# Autodesk Inventor assembly: Gantry Assembly R2
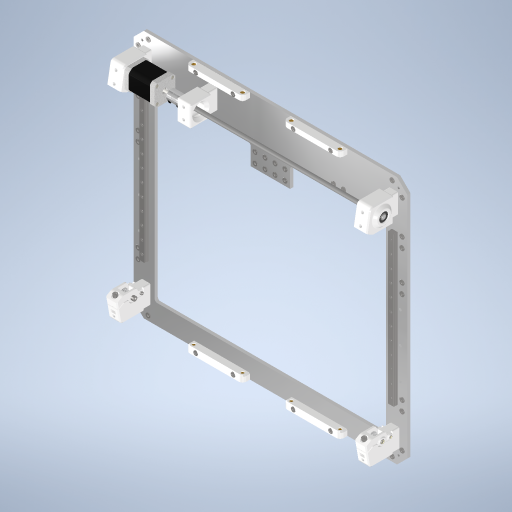
[picture p0: Inventor's stored thumbnail of the model, 512x512]
Saved by Autodesk Inventor 2024 (Build 280153000, 153)
## iProperties
Created: 2024-11-09
Part Number: Gantry Assembly R2
Document SubType Name: Assembly
Designer: Ishaan
Author: Ishaan
## Documents named in this file (24)
- E:\Projects\Axiom--IDEX-3D-Printer\CAD\04 - Gantry and Y-axis\Gantry Assembly R2.iam
- E:\Projects\Axiom--IDEX-3D-Printer\CAD\04 - Gantry and Y-axis\Printer Gantry Plate RevII.ipt
- E:\Projects\Axiom--IDEX-3D-Printer\CAD\00 - COTS Components\MGNR12 300mm Rail\MGNR12R100HM\MGNR12R100HM.ipt
- E:\Projects\Axiom--IDEX-3D-Printer\CAD\00 - COTS Components\Hardware\SHCSM3x8.ipt
- E:\Projects\Axiom--IDEX-3D-Printer\CAD\04 - Gantry and Y-axis\Y-axis Motor Block.ipt
- E:\Projects\Axiom--IDEX-3D-Printer\CAD\04 - Gantry and Y-axis\Y-axis Shaft Support.ipt
- E:\Projects\Axiom--IDEX-3D-Printer\CAD\04 - Gantry and Y-axis\Y-axis Bearing Pulley Block.ipt
- E:\Projects\Axiom--IDEX-3D-Printer\CAD\04 - Gantry and Y-axis\R2 Idler Block Left.ipt
- E:\Projects\Axiom--IDEX-3D-Printer\CAD\04 - Gantry and Y-axis\R2 Idler Block Right.ipt
- E:\Projects\Axiom--IDEX-3D-Printer\CAD\00 - COTS Components\NEMA 17 - Y-Axis\NEMA 17 Y-axis.ipt
- E:\Projects\Axiom--IDEX-3D-Printer\CAD\00 - COTS Components\9mm 20T GT2 Timing Pulley 5mm Bore\9mm 20T GT2 Timing Pulley 5mm Bore.ipt
- E:\Projects\Axiom--IDEX-3D-Printer\CAD\00 - COTS Components\9mm 20T GT2 Idler Pulley 5mm Bore\9mm 20T GT2 Idler Pulley 5mm Bore.ipt
- E:\Projects\Axiom--IDEX-3D-Printer\CAD\00 - COTS Components\608-2RS\608-2RS Bearing.ipt
- E:\Projects\Axiom--IDEX-3D-Printer\CAD\00 - COTS Components\9mm 20T GT2 Timing Pulley 8mm Bore\9mm 20T GT2 Timing Pulley 8mm Bore.ipt
- E:\Projects\Axiom--IDEX-3D-Printer\CAD\00 - COTS Components\5x8 Shaft Coupler\Flexible Coupling 5mm x 8mm.ipt
- E:\Projects\Axiom--IDEX-3D-Printer\CAD\00 - COTS Components\Hardware\SHCSM3x25.ipt
- E:\Projects\Axiom--IDEX-3D-Printer\CAD\00 - COTS Components\Hardware\SHCSM5x16.ipt
- E:\Projects\Axiom--IDEX-3D-Printer\CAD\00 - COTS Components\Hardware\Low Profile M5x12.ipt
- E:\Projects\Axiom--IDEX-3D-Printer\CAD\00 - COTS Components\Hardware\SHCSM5x25.ipt
- E:\Projects\Axiom--IDEX-3D-Printer\CAD\00 - COTS Components\Hardware\M5 LOCKNUT.ipt
- E:\Projects\Axiom--IDEX-3D-Printer\CAD\00 - COTS Components\Hardware\M3 LOCKNUT.ipt
- E:\Projects\Axiom--IDEX-3D-Printer\CAD\04 - Gantry and Y-axis\Y-axis Power Transfer Shaft 415mm.ipt
- E:\Projects\Axiom--IDEX-3D-Printer\CAD\04 - Gantry and Y-axis\Front Panel Mount.ipt
- E:\Projects\Axiom--IDEX-3D-Printer\CAD\00 - COTS Components\Hardware\M5 Heat Set Insert.ipt
## Components (118 placed, 23 different names)
1. Printer Gantry Plate RevII:1 — Insert:1, Insert:2, Insert:3, Insert:4, Insert:6, Insert:7, Insert:8, Insert:9, Insert:10, Insert:11, Insert:12, Insert:13, Insert:14, Insert:15, Insert:36, Insert:37, Insert:38, Insert:39, Insert:40, Insert:41, Insert:42, Insert:43, Insert:44, Insert:45, Insert:46, Insert:47, Insert:48, Insert:49, Insert:50, Insert:51, Insert:52, Insert:53, Insert:54, Insert:55, Insert:56, Insert:57, Insert:58, Insert:59, Insert:60, Insert:61, Insert:62, Insert:63, Insert:64, Insert:65, Insert:66, Insert:67, Insert:77, Insert:78, Insert:79, Insert:80, Insert:81, Insert:82, Insert:83, Insert:84
2. MGNR12R100HM:1 — Insert:3, Insert:4, Insert:5, Flush:3, Mate:4
3. MGNR12R100HM:2 — Insert:1, Insert:2, Flush:1, Flush:2, Insert:76
4. Y-axis Motor Block:1 — Insert:6, Insert:7, Insert:16, Insert:17, Insert:22, Insert:23, Insert:24, Insert:25, Insert:30, Insert:31
5. Y-axis Shaft Support:1 — Insert:8, Insert:9, Insert:18, Insert:32, Insert:33
6. Y-axis Bearing Pulley Block:1 — Insert:10, Insert:11, Insert:19, Insert:20, Insert:34, Insert:35
7. R2 Idler Block Left:1 — Insert:12, Insert:13, Mate:3, Insert:26, Insert:27, Insert:68, Mate:11, Mate:12, Insert:71, Insert:73, Angle:1, Insert:75, Angle:4
8. R2 Idler Block Right:1 — Insert:14, Insert:15, Mate:2, Insert:28, Insert:29, Insert:69, Mate:9, Mate:10, Insert:70, Insert:72, Angle:2, Insert:74, Angle:3
9. NEMA 17 Y-axis:1 — Insert:16, Insert:17, Mate:1, Insert:21
10. 9mm 20T GT2 Timing Pulley 5mm Bore:1 — Mate:1, Flush:1
11. 9mm 20T GT2 Idler Pulley 5mm Bore:1 — Mate:2, Flush:2
12. 9mm 20T GT2 Idler Pulley 5mm Bore:2 — Mate:3, Flush:3
13. 608-2RS Bearing:1 — Insert:18
14. 608-2RS Bearing:2 — Insert:20
15. 608-2RS Bearing:3 — Insert:19, Mate:5
16. 9mm 20T GT2 Timing Pulley 8mm Bore:1 — Mate:4, Mate:5
17. Y-axis Power Transfer Shaft 415mm:1
18. Flexible Coupling 5mm x 8mm:1 — Insert:21
19. Front Panel Mount:1 — Insert:77, Insert:79, Insert:85, Insert:86, Insert:94
20. Front Panel Mount:2 — Insert:78, Insert:80, Insert:87, Insert:88
21. Front Panel Mount:3 — Insert:81, Insert:82, Insert:91, Insert:92
22. Front Panel Mount:4 — Insert:83, Insert:84, Insert:89, Insert:90, Insert:93
23. SHCSM5x16:11 — Insert:85
24. SHCSM5x16:12 — Insert:86
25. SHCSM5x16:13 — Insert:87
26. SHCSM5x16:14 — Insert:88
27. SHCSM5x16:15 — Insert:89
28. SHCSM5x16:16 — Insert:90
29. SHCSM5x16:17 — Insert:91
30. SHCSM5x16:18 — Insert:92
31. SHCSM5x25:1 — Insert:68
32. SHCSM5x25:2 — Insert:69
33. SHCSM5x25:3 — Mate:9, Mate:10
34. SHCSM5x25:4 — Mate:11, Mate:12
35. SHCSM3x25:5 — Insert:70
36. SHCSM3x25:6 — Insert:71
37. M5 LOCKNUT:1 — Insert:72, Angle:2
38. M5 LOCKNUT:2 — Insert:73, Angle:1
39. M3 LOCKNUT:1 — Insert:74, Angle:3
40. M3 LOCKNUT:2 — Insert:75, Angle:4
41. Low Profile M5x12:1 — Insert:36
42. Low Profile M5x12:2 — Insert:37
43. Low Profile M5x12:3 — Insert:38
44. Low Profile M5x12:4 — Insert:39
45. Low Profile M5x12:5 — Insert:40
46. Low Profile M5x12:6 — Insert:41
47. Low Profile M5x12:7 — Insert:42
48. Low Profile M5x12:8 — Insert:43
49. Low Profile M5x12:9 — Insert:45
50. Low Profile M5x12:10 — Insert:46
51. Low Profile M5x12:11 — Insert:49
52. Low Profile M5x12:12 — Insert:50
53. Low Profile M5x12:13 — Insert:44
54. Low Profile M5x12:14 — Insert:47
55. Low Profile M5x12:15 — Insert:48
56. Low Profile M5x12:16 — Insert:51
57. Low Profile M5x12:17 — Insert:52
58. Low Profile M5x12:18 — Insert:53
59. Low Profile M5x12:19 — Insert:54
60. Low Profile M5x12:20 — Insert:55
61. Low Profile M5x12:21 — Insert:56
62. Low Profile M5x12:22 — Insert:57
63. Low Profile M5x12:23 — Insert:58
64. Low Profile M5x12:24 — Insert:59
65. Low Profile M5x12:25 — Insert:60
66. Low Profile M5x12:26 — Insert:61
67. Low Profile M5x12:27 — Insert:62
68. Low Profile M5x12:28 — Insert:63
69. Low Profile M5x12:29 — Insert:64
70. Low Profile M5x12:30 — Insert:65
71. Low Profile M5x12:31 — Insert:66
72. Low Profile M5x12:32 — Insert:67
73. SHCSM3x25:1 — Insert:22
74. SHCSM3x25:2 — Insert:23
75. SHCSM3x25:3 — Insert:24
76. SHCSM3x25:4 — Insert:25
77. SHCSM5x16:1 — Insert:26
78. SHCSM5x16:2 — Insert:27
79. SHCSM5x16:3 — Insert:28
80. SHCSM5x16:4 — Insert:29
81. SHCSM5x16:5 — Insert:30
82. SHCSM5x16:6 — Insert:31
83. SHCSM5x16:7 — Insert:32
84. SHCSM5x16:8 — Insert:33
85. SHCSM5x16:9 — Insert:34
86. SHCSM5x16:10 — Insert:35
87. M5 Heat Set Insert:2 — Insert:93
88. M5 Heat Set Insert:3
89. M5 Heat Set Insert:4
90. M5 Heat Set Insert:5
91. M5 Heat Set Insert:1 — Insert:94
92. M5 Heat Set Insert:6
93. M5 Heat Set Insert:7
94. M5 Heat Set Insert:8
95. SHCSM3x8:1 — Insert:76
96. SHCSM3x8:2
97. SHCSM3x8:3
98. SHCSM3x8:4
99. SHCSM3x8:5
100. SHCSM3x8:6
101. SHCSM3x8:7
102. SHCSM3x8:8
103. SHCSM3x8:9
104. SHCSM3x8:10
105. SHCSM3x8:11
106. SHCSM3x8:12
107. SHCSM3x8:13 — Insert:5
108. SHCSM3x8:14
109. SHCSM3x8:15
110. SHCSM3x8:16
111. SHCSM3x8:17
112. SHCSM3x8:18
113. SHCSM3x8:19
114. SHCSM3x8:20
115. SHCSM3x8:21
116. SHCSM3x8:22
117. SHCSM3x8:23
118. SHCSM3x8:24
## Component patterns: (4 elements, first: M5 Heat Set Insert:2), (4 elements, first: M5 Heat Set Insert:1), (12 elements, first: SHCSM3x8:1), (12 elements, first: SHCSM3x8:13)
## Relationships (113: Insert 94, Mate 12, Angle 4, Flush 3)
- Insert:1: Printer Gantry Plate RevII:1 ↔ MGNR12R100HM:2
- Insert:2: Printer Gantry Plate RevII:1 ↔ MGNR12R100HM:2
- Insert:3: Printer Gantry Plate RevII:1 ↔ MGNR12R100HM:1
- Insert:4: Printer Gantry Plate RevII:1 ↔ MGNR12R100HM:1
- Insert:5: MGNR12R100HM:1 ↔ SHCSM3x8:13
- Insert:6: Printer Gantry Plate RevII:1 ↔ Y-axis Motor Block:1
- Insert:7: Printer Gantry Plate RevII:1 ↔ Y-axis Motor Block:1
- Insert:8: Printer Gantry Plate RevII:1 ↔ Y-axis Shaft Support:1
- Insert:9: Printer Gantry Plate RevII:1 ↔ Y-axis Shaft Support:1
- Insert:10: Printer Gantry Plate RevII:1 ↔ Y-axis Bearing Pulley Block:1
- Insert:11: Printer Gantry Plate RevII:1 ↔ Y-axis Bearing Pulley Block:1
- Insert:12: Printer Gantry Plate RevII:1 ↔ R2 Idler Block Left:1
- Insert:13: Printer Gantry Plate RevII:1 ↔ R2 Idler Block Left:1
- Insert:14: Printer Gantry Plate RevII:1 ↔ R2 Idler Block Right:1
- Insert:15: Printer Gantry Plate RevII:1 ↔ R2 Idler Block Right:1
- Insert:16: Y-axis Motor Block:1 ↔ NEMA 17 Y-axis:1
- Insert:17: Y-axis Motor Block:1 ↔ NEMA 17 Y-axis:1
- Mate:1: NEMA 17 Y-axis:1 ↔ 9mm 20T GT2 Timing Pulley 5mm Bore:1
- Flush:1: MGNR12R100HM:2 ↔ 9mm 20T GT2 Timing Pulley 5mm Bore:1
- Mate:2: R2 Idler Block Right:1 ↔ 9mm 20T GT2 Idler Pulley 5mm Bore:1
- Mate:3: R2 Idler Block Left:1 ↔ 9mm 20T GT2 Idler Pulley 5mm Bore:2
- Flush:2: MGNR12R100HM:2 ↔ 9mm 20T GT2 Idler Pulley 5mm Bore:1
- Flush:3: MGNR12R100HM:1 ↔ 9mm 20T GT2 Idler Pulley 5mm Bore:2
- Insert:18: Y-axis Shaft Support:1 ↔ 608-2RS Bearing:1
- Insert:19: Y-axis Bearing Pulley Block:1 ↔ 608-2RS Bearing:3
- Insert:20: Y-axis Bearing Pulley Block:1 ↔ 608-2RS Bearing:2
- Mate:4: MGNR12R100HM:1 ↔ 9mm 20T GT2 Timing Pulley 8mm Bore:1
- Mate:5: 608-2RS Bearing:3 ↔ 9mm 20T GT2 Timing Pulley 8mm Bore:1
- [Mate]: 608-2RS Bearing:3 ↔ Y-axis Power Transfer Shaft 415mm:1
- [Mate]: 608-2RS Bearing:1 ↔ Y-axis Power Transfer Shaft 415mm:1
- [Mate] (1 mm): NEMA 17 Y-axis:1 ↔ Y-axis Power Transfer Shaft 415mm:1
- Insert:21 (-0.5 mm): NEMA 17 Y-axis:1 ↔ Flexible Coupling 5mm x 8mm:1
- Insert:22: Y-axis Motor Block:1 ↔ SHCSM3x25:1
- Insert:23: Y-axis Motor Block:1 ↔ SHCSM3x25:2
- Insert:24: Y-axis Motor Block:1 ↔ SHCSM3x25:3
- Insert:25: Y-axis Motor Block:1 ↔ SHCSM3x25:4
- Insert:26: R2 Idler Block Left:1 ↔ SHCSM5x16:1
- Insert:27: R2 Idler Block Left:1 ↔ SHCSM5x16:2
- Insert:28: R2 Idler Block Right:1 ↔ SHCSM5x16:3
- Insert:29: R2 Idler Block Right:1 ↔ SHCSM5x16:4
- Insert:30: Y-axis Motor Block:1 ↔ SHCSM5x16:5
- Insert:31: Y-axis Motor Block:1 ↔ SHCSM5x16:6
- Insert:32: Y-axis Shaft Support:1 ↔ SHCSM5x16:7
- Insert:33: Y-axis Shaft Support:1 ↔ SHCSM5x16:8
- Insert:34: Y-axis Bearing Pulley Block:1 ↔ SHCSM5x16:9
- Insert:35: Y-axis Bearing Pulley Block:1 ↔ SHCSM5x16:10
- Insert:36: Printer Gantry Plate RevII:1 ↔ Low Profile M5x12:1
- Insert:37: Printer Gantry Plate RevII:1 ↔ Low Profile M5x12:2
- Insert:38: Printer Gantry Plate RevII:1 ↔ Low Profile M5x12:3
- Insert:39: Printer Gantry Plate RevII:1 ↔ Low Profile M5x12:4
- Insert:40: Printer Gantry Plate RevII:1 ↔ Low Profile M5x12:5
- Insert:41: Printer Gantry Plate RevII:1 ↔ Low Profile M5x12:6
- Insert:42: Printer Gantry Plate RevII:1 ↔ Low Profile M5x12:7
- Insert:43: Printer Gantry Plate RevII:1 ↔ Low Profile M5x12:8
- Insert:44: Printer Gantry Plate RevII:1 ↔ Low Profile M5x12:13
- Insert:45: Printer Gantry Plate RevII:1 ↔ Low Profile M5x12:9
- Insert:46: Printer Gantry Plate RevII:1 ↔ Low Profile M5x12:10
- Insert:47: Printer Gantry Plate RevII:1 ↔ Low Profile M5x12:14
- Insert:48: Printer Gantry Plate RevII:1 ↔ Low Profile M5x12:15
- Insert:49: Printer Gantry Plate RevII:1 ↔ Low Profile M5x12:11
- Insert:50: Printer Gantry Plate RevII:1 ↔ Low Profile M5x12:12
- Insert:51: Printer Gantry Plate RevII:1 ↔ Low Profile M5x12:16
- Insert:52: Printer Gantry Plate RevII:1 ↔ Low Profile M5x12:17
- Insert:53: Printer Gantry Plate RevII:1 ↔ Low Profile M5x12:18
- Insert:54: Printer Gantry Plate RevII:1 ↔ Low Profile M5x12:19
- Insert:55: Printer Gantry Plate RevII:1 ↔ Low Profile M5x12:20
- Insert:56: Printer Gantry Plate RevII:1 ↔ Low Profile M5x12:21
- Insert:57: Printer Gantry Plate RevII:1 ↔ Low Profile M5x12:22
- Insert:58: Printer Gantry Plate RevII:1 ↔ Low Profile M5x12:23
- Insert:59: Printer Gantry Plate RevII:1 ↔ Low Profile M5x12:24
- Insert:60: Printer Gantry Plate RevII:1 ↔ Low Profile M5x12:25
- Insert:61: Printer Gantry Plate RevII:1 ↔ Low Profile M5x12:26
- Insert:62: Printer Gantry Plate RevII:1 ↔ Low Profile M5x12:27
- Insert:63: Printer Gantry Plate RevII:1 ↔ Low Profile M5x12:28
- Insert:64: Printer Gantry Plate RevII:1 ↔ Low Profile M5x12:29
- Insert:65: Printer Gantry Plate RevII:1 ↔ Low Profile M5x12:30
- Insert:66: Printer Gantry Plate RevII:1 ↔ Low Profile M5x12:31
- Insert:67: Printer Gantry Plate RevII:1 ↔ Low Profile M5x12:32
- Insert:68: R2 Idler Block Left:1 ↔ SHCSM5x25:1
- Insert:69: R2 Idler Block Right:1 ↔ SHCSM5x25:2
- Mate:9: R2 Idler Block Right:1 ↔ SHCSM5x25:3
- Mate:10: R2 Idler Block Right:1 ↔ SHCSM5x25:3
- Mate:11: R2 Idler Block Left:1 ↔ SHCSM5x25:4
- Mate:12: R2 Idler Block Left:1 ↔ SHCSM5x25:4
- Insert:70: R2 Idler Block Right:1 ↔ SHCSM3x25:5
- Insert:71: R2 Idler Block Left:1 ↔ SHCSM3x25:6
- Insert:72: R2 Idler Block Right:1 ↔ M5 LOCKNUT:1
- Insert:73: R2 Idler Block Left:1 ↔ M5 LOCKNUT:2
- Angle:1 (0 deg): R2 Idler Block Left:1 ↔ M5 LOCKNUT:2
- Angle:2 (0 deg): R2 Idler Block Right:1 ↔ M5 LOCKNUT:1
- Insert:74: R2 Idler Block Right:1 ↔ M3 LOCKNUT:1
- Angle:3 (0 deg): R2 Idler Block Right:1 ↔ M3 LOCKNUT:1
- Insert:75: R2 Idler Block Left:1 ↔ M3 LOCKNUT:2
- Angle:4 (0 deg): R2 Idler Block Left:1 ↔ M3 LOCKNUT:2
- Insert:76: MGNR12R100HM:2 ↔ SHCSM3x8:1
- Insert:77 (0.2 mm): Printer Gantry Plate RevII:1 ↔ Front Panel Mount:1
- Insert:78 (0.2 mm): Printer Gantry Plate RevII:1 ↔ Front Panel Mount:2
- Insert:79 (0.2 mm): Printer Gantry Plate RevII:1 ↔ Front Panel Mount:1
- Insert:80 (0.2 mm): Printer Gantry Plate RevII:1 ↔ Front Panel Mount:2
- Insert:81 (0.2 mm): Printer Gantry Plate RevII:1 ↔ Front Panel Mount:3
- Insert:82 (0.2 mm): Printer Gantry Plate RevII:1 ↔ Front Panel Mount:3
- Insert:83 (0.2 mm): Printer Gantry Plate RevII:1 ↔ Front Panel Mount:4
- Insert:84 (0.2 mm): Printer Gantry Plate RevII:1 ↔ Front Panel Mount:4
- Insert:85: Front Panel Mount:1 ↔ SHCSM5x16:11
- Insert:86: Front Panel Mount:1 ↔ SHCSM5x16:12
- Insert:87: Front Panel Mount:2 ↔ SHCSM5x16:13
- Insert:88: Front Panel Mount:2 ↔ SHCSM5x16:14
- Insert:89: Front Panel Mount:4 ↔ SHCSM5x16:15
- Insert:90: Front Panel Mount:4 ↔ SHCSM5x16:16
- Insert:91: Front Panel Mount:3 ↔ SHCSM5x16:17
- Insert:92: Front Panel Mount:3 ↔ SHCSM5x16:18
- Insert:93: Front Panel Mount:4 ↔ M5 Heat Set Insert:2
- Insert:94: Front Panel Mount:1 ↔ M5 Heat Set Insert:1
